# Autodesk Inventor assembly: 000.011 - Крепление по XT60 мама
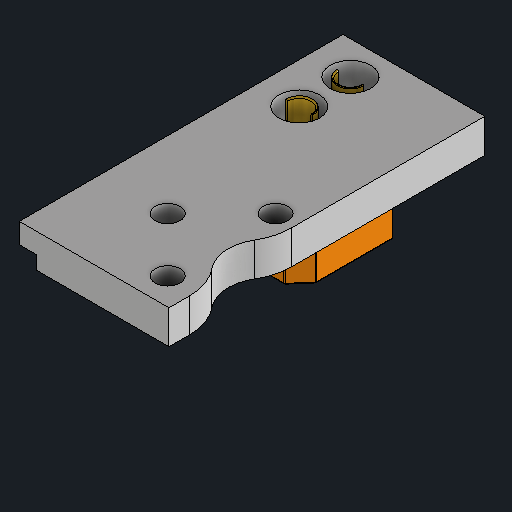
[picture p0: Inventor's stored thumbnail of the model, 512x512]
Saved by Autodesk Inventor 2025 (Build 290162000, 162)
## iProperties
Created: 2023-04-23
Part Number: 000.011 - Крепление по XT60 мама
Document SubType Name: Assembly
Designer: Иван Петров
Author: Иван Петров
## Documents named in this file (3)
- D:\Projects\OmniBot\design\000.003 - Крепление под XT60 мама.iam
- D:\Projects\OmniBot\design\000.003.001 - Основание.ipt
- D:\Projects\OmniBot\design\standart_components\XT60 Buchse.ipt
## Components (2 placed, 2 different names)
1. 000.003.001 - Основание:1 — Совмещение:2, Совмещение:3, Совмещение:4
2. XT60 Buchse:1 — Совмещение:2, Совмещение:3, Совмещение:4
## Relationships (3: Mate 3)
- Совмещение:2 [Mate]: 000.003.001 - Основание:1 ↔ XT60 Buchse:1
- Совмещение:3 [Mate]: 000.003.001 - Основание:1 ↔ XT60 Buchse:1
- Совмещение:4 [Mate]: 000.003.001 - Основание:1 ↔ XT60 Buchse:1
